# Autodesk Inventor assembly: s-assy-ring_gear
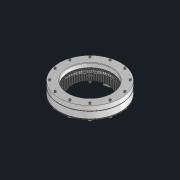
[picture p0: Inventor's stored thumbnail of the model, 180x180]
Saved by Autodesk Inventor 2021 (Build 250183000, 183)
## iProperties
Created: 2021-07-12
Part Number: s-assy-ring_gear
Document SubType Name: Assembly
Designer: yuta0
Mass: 180.782 g
Surface Area: 832.349 cm^2
Volume: 122.833 cm^3
Density: 1.47176 g/cm^3
Author: yuta0
## Documents named in this file (10)
- C:\Users\yuta0\Documents\GitHub\catchrobo_hardware\assy-robot\s-assy-ring_gear.iam
- C:\Users\yuta0\Documents\GitHub\catchrobo_hardware\assy-robot\base33.ipt
- C:\Users\yuta0\Documents\GitHub\catchrobo_hardware\assy-robot\carbon_plate13.ipt
- C:\Users\yuta0\Documents\GitHub\catchrobo_hardware\assy-robot\CB4-30.ipt
- C:\Users\yuta0\Documents\GitHub\catchrobo_hardware\assy-robot\base26.ipt
- C:\Users\yuta0\Documents\GitHub\catchrobo_hardware\assy-robot\carbon_plate9.ipt
- C:\Users\yuta0\Documents\GitHub\catchrobo_hardware\assy-robot\SS-5GL.iam
- C:\Users\yuta0\Documents\GitHub\catchrobo_hardware\assy-robot\CB2-10.ipt
- C:\Users\yuta0\Documents\GitHub\catchrobo_hardware\assy-robot\LBNR2.ipt
- C:\Users\yuta0\Documents\GitHub\catchrobo_hardware\assy-robot\CBSTSR4-14.ipt
## Components (25 placed, 9 different names)
1. base33:1 — フラッシュ:2, メイト:5, メイト:6, メイト:11, メイト:29, メイト:41
2. base26:1 — メイト:11, メイト:12, メイト:31
3. carbon_plate13:1 — メイト:4, メイト:5, メイト:6, メイト:12
4. carbon_plate9:1 — メイト:30, メイト:32, メイト:38, メイト:39, メイト:40, メイト:41, メイト:42, メイト:43, メイト:48, メイト:49, メイト:50
5. SS-5GL:2 [sub-assembly] — メイト:38, メイト:39, メイト:40, メイト:45
6. CB4-30:1 — メイト:29, メイト:30
7. CB4-30:2
8. CB4-30:3
9. CB4-30:4
10. CB4-30:5
11. CB4-30:6 — メイト:42
12. CB4-30:7
13. CB4-30:8
14. CB4-30:9
15. CB4-30:10
16. CB4-30:11
17. CB4-30:12
18. CB2-10:1 — メイト:43, メイト:45, メイト:47
19. LBNR2:1 — メイト:47, メイト:48
20. CB2-10:2
21. LBNR2:2
22. CBSTSR4-14:1 — メイト:49, メイト:50
23. CBSTSR4-14:2
24. CBSTSR4-14:3
25. CBSTSR4-14:4
## Component patterns: (12 elements, first: CB4-30:1), (2 elements, first: CB2-10:1 + LBNR2:1), (4 elements, first: CBSTSR4-14:1)
## Relationships (21: Mate 20, Flush 1)
- フラッシュ:2 [Flush]: base33:1
- メイト:4 [Mate]: carbon_plate13:1
- メイト:5 [Mate]: base33:1 ↔ carbon_plate13:1
- メイト:6 [Mate]: base33:1 ↔ carbon_plate13:1
- メイト:11 [Mate]: base33:1 ↔ base26:1
- メイト:12 [Mate]: base26:1 ↔ carbon_plate13:1
- メイト:29 [Mate]: base33:1 ↔ CB4-30:1
- メイト:30 [Mate]: carbon_plate9:1 ↔ CB4-30:1
- メイト:31 [Mate]: base26:1
- メイト:32 [Mate]: carbon_plate9:1
- メイト:38 [Mate]: carbon_plate9:1 ↔ SS-5GL:2
- メイト:39 [Mate]: carbon_plate9:1 ↔ SS-5GL:2
- メイト:40 [Mate]: carbon_plate9:1 ↔ SS-5GL:2
- メイト:41 [Mate]: base33:1 ↔ carbon_plate9:1
- メイト:42 [Mate]: carbon_plate9:1 ↔ CB4-30:6
- メイト:43 [Mate]: carbon_plate9:1 ↔ CB2-10:1
- メイト:45 [Mate]: SS-5GL:2 ↔ CB2-10:1
- メイト:47 [Mate]: CB2-10:1 ↔ LBNR2:1
- メイト:48 [Mate]: carbon_plate9:1 ↔ LBNR2:1
- メイト:49 [Mate]: carbon_plate9:1 ↔ CBSTSR4-14:1
- メイト:50 [Mate]: carbon_plate9:1 ↔ CBSTSR4-14:1
